# Autodesk Inventor assembly: ASY GBK центральная стенка
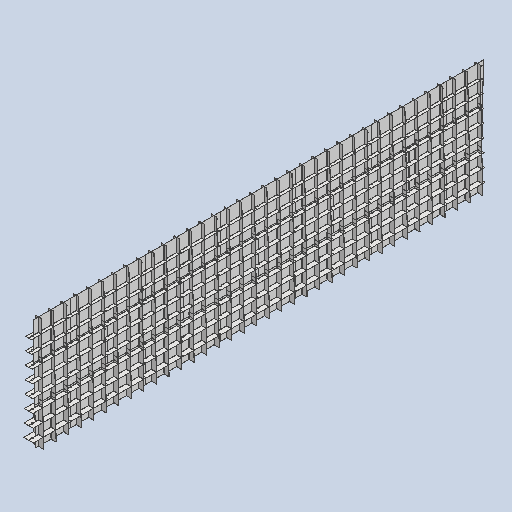
[picture p0: Inventor's stored thumbnail of the model, 512x512]
Saved by Autodesk Inventor 2026 (Build 300175000, 175)
## iProperties
Created: 2026-05-28
Part Number: ASY GBK центральная стенка
Document SubType Name: Assembly
Designer: pokla
Author: pokla
## Documents named in this file (10)
- C:\Users\pokla\Documents\Inventor\GBK-Gubkinskiy\ASY GBK центральная стенка.iam
- C:\Users\pokla\Documents\Inventor\GBK-Gubkinskiy\ASY GBK 3110 central wall shield 1.iam
- C:\Users\pokla\Documents\Inventor\GBK-Gubkinskiy\ASY GBK 3120 central wall shield 2.iam
- C:\Users\pokla\Documents\Inventor\GBK-Gubkinskiy\ASY GBK 3210 central wall shield 4.iam
- C:\Users\pokla\Documents\Inventor\GBK-Gubkinskiy\ASY GBK 3220 central wall shield 5.iam
- C:\Users\pokla\Documents\Inventor\GBK-Gubkinskiy\ASY GBK 3310 central wall shield 7.iam
- C:\Users\pokla\Documents\Inventor\GBK-Gubkinskiy\ASY GBK 3320 central wall shield 8.iam
- C:\Users\pokla\Documents\Inventor\GBK-Gubkinskiy\ASY GBK 3330 central wall shield 9.iam
- C:\Users\pokla\Documents\Inventor\GBK-Gubkinskiy\ASY GBK 3230 central wall shield 6.iam
- C:\Users\pokla\Documents\Inventor\GBK-Gubkinskiy\ASY GBK 3130 central wall shield 3.iam
## Components (20 placed, 12 different names)
1. ASY GBK 3110 central wall shield 1.iam:1 [sub-assembly] — Совмещение:1, Жесткий:1, Совмещение:4, Совмещение:5, Заподлицо:1, Совмещение:6
2. ASY GBK 3120 central wall shield 2.iam:1 [sub-assembly] — Жесткий:1, Жесткий:6
3. ASY GBK 3210 central wall shield 4.iam:1 [sub-assembly] — Жесткий:3, Совмещение:5, Заподлицо:1, Совмещение:6, Совмещение:7, Заподлицо:2, Совмещение:8
4. ASY GBK 3220 central wall shield 5.iam:1 [sub-assembly] — Жесткий:3, Жесткий:11
5. ASY GBK 3310 central wall shield 7.iam:1 [sub-assembly] — Жесткий:5, Совмещение:7, Заподлицо:2, Совмещение:8
6. ASY GBK 3320 central wall shield 8.iam:1 [sub-assembly] — Жесткий:5, Жесткий:15
7. ASY GBK 3330 central wall shield 9.iam:1 [sub-assembly] — Жесткий:19
8. ASY GBK 3230 central wall shield 6.iam:1 [sub-assembly] — Жесткий:14
9. ASY GBK 3130 central wall shield 3.iam:1 [sub-assembly] — Жесткий:10
10. ASY GBK 3120 central wall shield 2:2 [sub-assembly] — Жесткий:6, Жесткий:7
11. ASY GBK 3120 central wall shield 2:3 [sub-assembly] — Жесткий:7, Жесткий:8
12. ASY GBK 3120 central wall shield 2:4 [sub-assembly] — Жесткий:8, Жесткий:9
13. ASY GBK 3120 central wall shield 2:5 [sub-assembly] — Жесткий:9, Жесткий:10
14. ASY GBK 3220 central wall shield 4:2 [sub-assembly] — Жесткий:11, Жесткий:12
15. ASY GBK 3220 central wall shield 4:3 [sub-assembly] — Жесткий:12, Жесткий:13
16. ASY GBK 3220 central wall shield 4:4 [sub-assembly] — Жесткий:13, Жесткий:14
17. ASY GBK 3320 central wall shield 8:2 [sub-assembly] — Жесткий:15, Жесткий:16
18. ASY GBK 3320 central wall shield 8:3 [sub-assembly] — Жесткий:16, Жесткий:17
19. ASY GBK 3320 central wall shield 8:4 [sub-assembly] — Жесткий:17, Жесткий:18
20. ASY GBK 3320 central wall shield 8:5 [sub-assembly] — Жесткий:18, Жесткий:19
## Relationships (25: WeldJoint 17, Mate 6, Flush 2)
- Совмещение:1 [Mate]: ASY GBK 3110 central wall shield 1.iam:1
- Жесткий:1 [WeldJoint] (1 mm): ASY GBK 3110 central wall shield 1.iam:1 ↔ ASY GBK 3120 central wall shield 2.iam:1
- Совмещение:4 [Mate]: ASY GBK 3110 central wall shield 1.iam:1
- Жесткий:3 [WeldJoint] (1 mm): ASY GBK 3210 central wall shield 4.iam:1 ↔ ASY GBK 3220 central wall shield 5.iam:1
- Жесткий:5 [WeldJoint] (1 mm): ASY GBK 3310 central wall shield 7.iam:1 ↔ ASY GBK 3320 central wall shield 8.iam:1
- Жесткий:6 [WeldJoint] (1 mm): ASY GBK 3120 central wall shield 2.iam:1 ↔ ASY GBK 3120 central wall shield 2:2
- Жесткий:7 [WeldJoint] (1 mm): ASY GBK 3120 central wall shield 2:2 ↔ ASY GBK 3120 central wall shield 2:3
- Жесткий:8 [WeldJoint] (1 mm): ASY GBK 3120 central wall shield 2:3 ↔ ASY GBK 3120 central wall shield 2:4
- Жесткий:9 [WeldJoint] (1 mm): ASY GBK 3120 central wall shield 2:4 ↔ ASY GBK 3120 central wall shield 2:5
- Жесткий:10 [WeldJoint] (1 mm): ASY GBK 3130 central wall shield 3.iam:1 ↔ ASY GBK 3120 central wall shield 2:5
- Жесткий:11 [WeldJoint] (1 mm): ASY GBK 3220 central wall shield 5.iam:1 ↔ ASY GBK 3220 central wall shield 4:2
- Жесткий:12 [WeldJoint] (1 mm): ASY GBK 3220 central wall shield 4:2 ↔ ASY GBK 3220 central wall shield 4:3
- Жесткий:13 [WeldJoint] (1 mm): ASY GBK 3220 central wall shield 4:3 ↔ ASY GBK 3220 central wall shield 4:4
- Жесткий:14 [WeldJoint] (1 mm): ASY GBK 3230 central wall shield 6.iam:1 ↔ ASY GBK 3220 central wall shield 4:4
- Жесткий:15 [WeldJoint] (1 mm): ASY GBK 3320 central wall shield 8.iam:1 ↔ ASY GBK 3320 central wall shield 8:2
- Жесткий:16 [WeldJoint] (1 mm): ASY GBK 3320 central wall shield 8:2 ↔ ASY GBK 3320 central wall shield 8:3
- Жесткий:17 [WeldJoint] (1 mm): ASY GBK 3320 central wall shield 8:3 ↔ ASY GBK 3320 central wall shield 8:4
- Жесткий:18 [WeldJoint] (1 mm): ASY GBK 3320 central wall shield 8:4 ↔ ASY GBK 3320 central wall shield 8:5
- Жесткий:19 [WeldJoint] (1 mm): ASY GBK 3330 central wall shield 9.iam:1 ↔ ASY GBK 3320 central wall shield 8:5
- Совмещение:5 [Mate] (1 mm): ASY GBK 3110 central wall shield 1.iam:1 ↔ ASY GBK 3210 central wall shield 4.iam:1
- Заподлицо:1 [Flush]: ASY GBK 3110 central wall shield 1.iam:1 ↔ ASY GBK 3210 central wall shield 4.iam:1
- Совмещение:6 [Mate] (1 mm): ASY GBK 3110 central wall shield 1.iam:1 ↔ ASY GBK 3210 central wall shield 4.iam:1
- Совмещение:7 [Mate] (1 mm): ASY GBK 3210 central wall shield 4.iam:1 ↔ ASY GBK 3310 central wall shield 7.iam:1
- Заподлицо:2 [Flush]: ASY GBK 3210 central wall shield 4.iam:1 ↔ ASY GBK 3310 central wall shield 7.iam:1
- Совмещение:8 [Mate] (1 mm): ASY GBK 3210 central wall shield 4.iam:1 ↔ ASY GBK 3310 central wall shield 7.iam:1
